# Autodesk Inventor assembly: Press
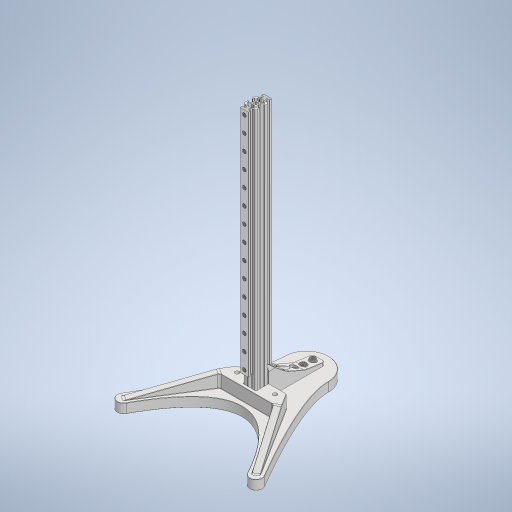
[picture p0: Inventor's stored thumbnail of the model, 512x512]
Saved by Autodesk Inventor 2024 (Build 280153000, 153)
## iProperties
Created: 2023-12-26
Part Number: Press
Document SubType Name: Assembly
Designer: denni
Author: denni
## Documents named in this file (8)
- D:\GIT\ThreadedInsertPress\Press.iam
- D:\GIT\ThreadedInsertPress\AluminiumTSlotProfil20x20x420.ipt
- D:\GIT\ThreadedInsertPress\PressBase.ipt
- D:\GIT\ThreadedInsertPress\TS_04_12_364.ipt
- D:\Inventor\Content Center Files\R2024\de-DE\ISO 4762(1)\DIN EN ISO 4762 - M3 x 10.ipt
- D:\GIT\ThreadedInsertPress\BraketBack.ipt
- D:\Inventor\Content Center Files\R2024\de-DE\ISO 4762(1)\DIN EN ISO 4762 - M5 x 16.ipt
- D:\Inventor\Content Center Files\R2024\de-DE\ISO 4762(1)\DIN EN ISO 4762 - M5 x 10.ipt
## Components (40 placed, 7 different names)
1. AluminiumTSlotProfil20x20x420:1 — Passend:1, Passend:2, Fluchtend:1, Fluchtend:2, Passend:3, Passend:4, Fluchtend:3, Fluchtend:4, Fluchtend:5
2. PressBase:1 — Passend:1, Passend:2, Fluchtend:1, Passend:5, Passend:6, Passend:7
3. TS_04_12_364:1 — Fluchtend:2, Passend:3, Fluchtend:5, Einfügen:1, Einfügen:2, Einfügen:3, Einfügen:4, Einfügen:5, Einfügen:6, Einfügen:7, Einfügen:8, Einfügen:9, Einfügen:10, Einfügen:11, Einfügen:12, Einfügen:13, Einfügen:14, Einfügen:15
4. TS_04_12_364:2 — Passend:4, Fluchtend:3, Fluchtend:4, Einfügen:16, Einfügen:17, Einfügen:18, Einfügen:19, Einfügen:20, Einfügen:21, Einfügen:22, Einfügen:23, Einfügen:24, Einfügen:25, Einfügen:26, Einfügen:27, Einfügen:28, Einfügen:29, Einfügen:30
5. DIN EN ISO 4762 M3 x 10:1 — Einfügen:1
6. DIN EN ISO 4762 M3 x 10:2 — Einfügen:2
7. DIN EN ISO 4762 M3 x 10:3 — Einfügen:3
8. DIN EN ISO 4762 M3 x 10:4 — Einfügen:4
9. DIN EN ISO 4762 M3 x 10:5 — Einfügen:5
10. DIN EN ISO 4762 M3 x 10:6 — Einfügen:6
11. DIN EN ISO 4762 M3 x 10:7 — Einfügen:7
12. DIN EN ISO 4762 M3 x 10:8 — Einfügen:8
13. DIN EN ISO 4762 M3 x 10:9 — Einfügen:9
14. DIN EN ISO 4762 M3 x 10:10 — Einfügen:10
15. DIN EN ISO 4762 M3 x 10:11 — Einfügen:11
16. DIN EN ISO 4762 M3 x 10:12 — Einfügen:12
17. DIN EN ISO 4762 M3 x 10:13 — Einfügen:13
18. DIN EN ISO 4762 M3 x 10:14 — Einfügen:14
19. DIN EN ISO 4762 M3 x 10:15 — Einfügen:15
20. DIN EN ISO 4762 M3 x 10:16 — Einfügen:16
21. DIN EN ISO 4762 M3 x 10:17 — Einfügen:17
22. DIN EN ISO 4762 M3 x 10:18 — Einfügen:18
23. DIN EN ISO 4762 M3 x 10:19 — Einfügen:19
24. DIN EN ISO 4762 M3 x 10:20 — Einfügen:20
25. DIN EN ISO 4762 M3 x 10:21 — Einfügen:21
26. DIN EN ISO 4762 M3 x 10:22 — Einfügen:22
27. DIN EN ISO 4762 M3 x 10:23 — Einfügen:23
28. DIN EN ISO 4762 M3 x 10:24 — Einfügen:24
29. DIN EN ISO 4762 M3 x 10:25 — Einfügen:25
30. DIN EN ISO 4762 M3 x 10:26 — Einfügen:26
31. DIN EN ISO 4762 M3 x 10:27 — Einfügen:27
32. DIN EN ISO 4762 M3 x 10:28 — Einfügen:28
33. DIN EN ISO 4762 M3 x 10:29 — Einfügen:29
34. DIN EN ISO 4762 M3 x 10:30 — Einfügen:30
35. BraketBack:1 — Passend:5, Passend:6, Passend:7, Einfügen:31, Einfügen:32, Einfügen:33, Einfügen:34, Einfügen:35
36. DIN EN ISO 4762 M5 x 16:1 — Einfügen:31
37. DIN EN ISO 4762 M5 x 16:2 — Einfügen:32
38. DIN EN ISO 4762 M5 x 16:3 — Einfügen:33
39. DIN EN ISO 4762 M5 x 10:1 — Einfügen:34
40. DIN EN ISO 4762 M5 x 10:2 — Einfügen:35
## Relationships (47: Insert 35, Mate 7, Flush 5)
- Passend:1 [Mate] (0.5 mm): AluminiumTSlotProfil20x20x420:1 ↔ PressBase:1
- Passend:2 [Mate] (0.5 mm): AluminiumTSlotProfil20x20x420:1 ↔ PressBase:1
- Fluchtend:1 [Flush]: AluminiumTSlotProfil20x20x420:1 ↔ PressBase:1
- Fluchtend:2 [Flush] (-4 mm): AluminiumTSlotProfil20x20x420:1 ↔ TS_04_12_364:1
- Passend:3 [Mate]: AluminiumTSlotProfil20x20x420:1 ↔ TS_04_12_364:1
- Passend:4 [Mate]: AluminiumTSlotProfil20x20x420:1 ↔ TS_04_12_364:2
- Fluchtend:3 [Flush] (4 mm): AluminiumTSlotProfil20x20x420:1 ↔ TS_04_12_364:2
- Fluchtend:4 [Flush]: AluminiumTSlotProfil20x20x420:1 ↔ TS_04_12_364:2
- Fluchtend:5 [Flush]: AluminiumTSlotProfil20x20x420:1 ↔ TS_04_12_364:1
- Einfügen:1 [Insert]: TS_04_12_364:1 ↔ DIN EN ISO 4762 M3 x 10:1
- Einfügen:2 [Insert]: TS_04_12_364:1 ↔ DIN EN ISO 4762 M3 x 10:2
- Einfügen:3 [Insert]: TS_04_12_364:1 ↔ DIN EN ISO 4762 M3 x 10:3
- Einfügen:4 [Insert]: TS_04_12_364:1 ↔ DIN EN ISO 4762 M3 x 10:4
- Einfügen:5 [Insert]: TS_04_12_364:1 ↔ DIN EN ISO 4762 M3 x 10:5
- Einfügen:6 [Insert]: TS_04_12_364:1 ↔ DIN EN ISO 4762 M3 x 10:6
- Einfügen:7 [Insert]: TS_04_12_364:1 ↔ DIN EN ISO 4762 M3 x 10:7
- Einfügen:8 [Insert]: TS_04_12_364:1 ↔ DIN EN ISO 4762 M3 x 10:8
- Einfügen:9 [Insert]: TS_04_12_364:1 ↔ DIN EN ISO 4762 M3 x 10:9
- Einfügen:10 [Insert]: TS_04_12_364:1 ↔ DIN EN ISO 4762 M3 x 10:10
- Einfügen:11 [Insert]: TS_04_12_364:1 ↔ DIN EN ISO 4762 M3 x 10:11
- Einfügen:12 [Insert]: TS_04_12_364:1 ↔ DIN EN ISO 4762 M3 x 10:12
- Einfügen:13 [Insert]: TS_04_12_364:1 ↔ DIN EN ISO 4762 M3 x 10:13
- Einfügen:14 [Insert]: TS_04_12_364:1 ↔ DIN EN ISO 4762 M3 x 10:14
- Einfügen:15 [Insert]: TS_04_12_364:1 ↔ DIN EN ISO 4762 M3 x 10:15
- Einfügen:16 [Insert]: TS_04_12_364:2 ↔ DIN EN ISO 4762 M3 x 10:16
- Einfügen:17 [Insert]: TS_04_12_364:2 ↔ DIN EN ISO 4762 M3 x 10:17
- Einfügen:18 [Insert]: TS_04_12_364:2 ↔ DIN EN ISO 4762 M3 x 10:18
- Einfügen:19 [Insert]: TS_04_12_364:2 ↔ DIN EN ISO 4762 M3 x 10:19
- Einfügen:20 [Insert]: TS_04_12_364:2 ↔ DIN EN ISO 4762 M3 x 10:20
- Einfügen:21 [Insert]: TS_04_12_364:2 ↔ DIN EN ISO 4762 M3 x 10:21
- Einfügen:22 [Insert]: TS_04_12_364:2 ↔ DIN EN ISO 4762 M3 x 10:22
- Einfügen:23 [Insert]: TS_04_12_364:2 ↔ DIN EN ISO 4762 M3 x 10:23
- Einfügen:24 [Insert]: TS_04_12_364:2 ↔ DIN EN ISO 4762 M3 x 10:24
- Einfügen:25 [Insert]: TS_04_12_364:2 ↔ DIN EN ISO 4762 M3 x 10:25
- Einfügen:26 [Insert]: TS_04_12_364:2 ↔ DIN EN ISO 4762 M3 x 10:26
- Einfügen:27 [Insert]: TS_04_12_364:2 ↔ DIN EN ISO 4762 M3 x 10:27
- Einfügen:28 [Insert]: TS_04_12_364:2 ↔ DIN EN ISO 4762 M3 x 10:28
- Einfügen:29 [Insert]: TS_04_12_364:2 ↔ DIN EN ISO 4762 M3 x 10:29
- Einfügen:30 [Insert]: TS_04_12_364:2 ↔ DIN EN ISO 4762 M3 x 10:30
- Passend:5 [Mate]: PressBase:1 ↔ BraketBack:1
- Passend:6 [Mate]: PressBase:1 ↔ BraketBack:1
- Passend:7 [Mate]: PressBase:1 ↔ BraketBack:1
- Einfügen:31 [Insert]: BraketBack:1 ↔ DIN EN ISO 4762 M5 x 16:1
- Einfügen:32 [Insert]: BraketBack:1 ↔ DIN EN ISO 4762 M5 x 16:2
- Einfügen:33 [Insert]: BraketBack:1 ↔ DIN EN ISO 4762 M5 x 16:3
- Einfügen:34 [Insert]: BraketBack:1 ↔ DIN EN ISO 4762 M5 x 10:1
- Einfügen:35 [Insert]: BraketBack:1 ↔ DIN EN ISO 4762 M5 x 10:2
